# Autodesk Inventor assembly: Cross Bar Assembly
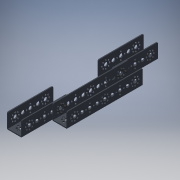
[picture p0: Inventor's stored thumbnail of the model, 180x180]
Saved by Autodesk Inventor 2016 (Build 200138000, 138)
## iProperties
Created: 2015-09-08
Part Number: Cross Bar Assembly
Document SubType Name: Assembly
Designer: phiro
Author: phiro
## Documents named in this file (4)
- C:\Users\phiro\Documents\GitHub\phi_robotics\3d-models\FTC_Tetrix_KOP_Block_Party\Tim Bloot Designs\Tutorial Bot\Cross Bar Assembly.iam
- C:\Users\phiro\Documents\GitHub\phi_robotics\3d-models\FTC_Tetrix_KOP_Block_Party\Tetrix_Kit_FTC\Autodesk Inventor Files\tetrix_c_channel-2.ipt
- C:\Users\phiro\Documents\GitHub\phi_robotics\3d-models\FTC_Tetrix_KOP_Block_Party\Tetrix_Kit_FTC\Autodesk Inventor Files\tetrix_c_channel-3.ipt
- C:\Users\phiro\Documents\GitHub\phi_robotics\3d-models\FTC_Tetrix_KOP_Block_Party\Tetrix_Kit_FTC\Autodesk Inventor Files\tetrix_screw-short.ipt
## Components (11 placed, 3 different names)
1. tetrix_c_channel-2:2 — Rigid:1, Rotational:1, Rotational:2, Rotational:3, Rotational:4
2. tetrix_c_channel-2:3 — Rigid:2, Rotational:5, Rotational:6, Rotational:7, Rotational:8
3. tetrix_c_channel-3:1 — Rigid:1, Rigid:2
4. tetrix_screw-short:2 — Rotational:5
5. tetrix_screw-short:3 — Rotational:7
6. tetrix_screw-short:4 — Rotational:8
7. tetrix_screw-short:5 — Rotational:6
8. tetrix_screw-short:6 — Rotational:4
9. tetrix_screw-short:7 — Rotational:3
10. tetrix_screw-short:8 — Rotational:1
11. tetrix_screw-short:9 — Rotational:2
## Relationships (10: RevoluteJoint 8, WeldJoint 2)
- Rigid:1 [WeldJoint]: tetrix_c_channel-2:2 ↔ tetrix_c_channel-3:1
- Rigid:2 [WeldJoint]: tetrix_c_channel-2:3 ↔ tetrix_c_channel-3:1
- Rotational:1 [RevoluteJoint]: tetrix_c_channel-2:2 ↔ tetrix_screw-short:8
- Rotational:2 [RevoluteJoint]: tetrix_c_channel-2:2 ↔ tetrix_screw-short:9
- Rotational:3 [RevoluteJoint]: tetrix_c_channel-2:2 ↔ tetrix_screw-short:7
- Rotational:4 [RevoluteJoint]: tetrix_c_channel-2:2 ↔ tetrix_screw-short:6
- Rotational:5 [RevoluteJoint]: tetrix_c_channel-2:3 ↔ tetrix_screw-short:2
- Rotational:6 [RevoluteJoint]: tetrix_c_channel-2:3 ↔ tetrix_screw-short:5
- Rotational:7 [RevoluteJoint]: tetrix_c_channel-2:3 ↔ tetrix_screw-short:3
- Rotational:8 [RevoluteJoint]: tetrix_c_channel-2:3 ↔ tetrix_screw-short:4
